# Autodesk Inventor assembly: Hilfsbaugruppe Vibrationsdämpfung
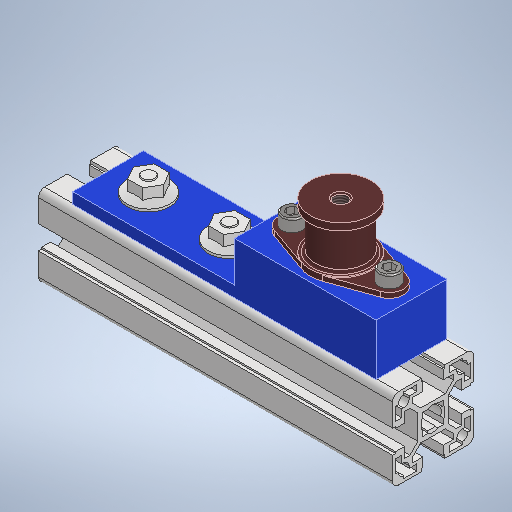
[picture p0: Inventor's stored thumbnail of the model, 512x512]
Saved by Autodesk Inventor 2025.2 (Build 292293000, 293)
## iProperties
Created: 2025-06-22
Part Number: Hilfsbaugruppe Vibrationsdämpfung
Document SubType Name: Assembly
Designer: Jakob
Author: Jakob
## Documents named in this file (6)
- D:\Useless_Box\CAD-Paspa\Useless Box\Zeichnung_JH\Hilfsbaugruppe Vibrationsdämpfung.iam
- D:\Useless_Box\CAD-Paspa\Useless Box\Eigene Bauteile\Vibrationsdaempfer\Rexroth_Profil_40x40_2175_8.ipt
- D:\Useless_Box\CAD-Paspa\Useless Box\Eigene Bauteile\Vibrationsdaempfer\Adapterplatte_Vibrationsdaempfer.ipt
- D:\Useless_Box\CAD-Paspa\Useless Box\Eigene Bauteile\Vibrationsdaempfer\AIS2024\NHF19-3026-M8.ipt
- D:\Useless_Box\CAD-Paspa\Useless Box\Standart Bauteile\ISO 4762 - M6 x 12ISO.ipt
- D:\Useless_Box\CAD-Paspa\Useless Box\Eigene Bauteile\Vibrationsdaempfer\Rexroth_Schraube_Mutter_modifiziert_fuer_daempfer.iam
## Components (7 placed, 5 different names)
1. Rexroth_Profil_40x40_2175_8:1 — Passend:1, Passend:2, Fluchtend:1, Fluchtend:4, Passend:10
2. Adapterplatte_Vibrationsdaempfer:1 — Passend:7, Fluchtend:4, Fluchtend:6, Passend:8, Passend:9, Passend:19, Passend:20, Fluchtend:7, Passend:21, Passend:22, Passend:23
3. NHF19-3026-M8:1 — Fluchtend:6, Passend:8, Passend:9, Passend:10, Passend:11, Passend:12, Passend:13, Passend:14
4. ISO 4762 - M6 x 12ISO:1 — Passend:12, Passend:14
5. ISO 4762 - M6 x 12ISO:2 — Passend:11, Passend:13
6. Rexroth_Schraube_Mutter_modifiziert_fuer_daempfer:1 [sub-assembly] — Fluchtend:7, Passend:21, Passend:23
7. Rexroth_Schraube_Mutter_modifiziert_fuer_daempfer:2 [sub-assembly] — Passend:19, Passend:20, Passend:22
## Relationships (19: Mate 15, Flush 4)
- Passend:1 [Mate]: Rexroth_Profil_40x40_2175_8:1
- Passend:2 [Mate]: Rexroth_Profil_40x40_2175_8:1
- Fluchtend:1 [Flush]: Rexroth_Profil_40x40_2175_8:1
- Passend:7 [Mate]: Adapterplatte_Vibrationsdaempfer:1
- Fluchtend:4 [Flush]: Rexroth_Profil_40x40_2175_8:1 ↔ Adapterplatte_Vibrationsdaempfer:1
- Fluchtend:6 [Flush]: Adapterplatte_Vibrationsdaempfer:1 ↔ NHF19-3026-M8:1
- Passend:8 [Mate]: Adapterplatte_Vibrationsdaempfer:1 ↔ NHF19-3026-M8:1
- Passend:9 [Mate]: Adapterplatte_Vibrationsdaempfer:1 ↔ NHF19-3026-M8:1
- Passend:10 [Mate] (45.642 mm): Rexroth_Profil_40x40_2175_8:1 ↔ NHF19-3026-M8:1
- Passend:11 [Mate]: NHF19-3026-M8:1 ↔ ISO 4762 - M6 x 12ISO:2
- Passend:12 [Mate]: NHF19-3026-M8:1 ↔ ISO 4762 - M6 x 12ISO:1
- Passend:13 [Mate]: NHF19-3026-M8:1 ↔ ISO 4762 - M6 x 12ISO:2
- Passend:14 [Mate]: NHF19-3026-M8:1 ↔ ISO 4762 - M6 x 12ISO:1
- Passend:19 [Mate]: Adapterplatte_Vibrationsdaempfer:1 ↔ Rexroth_Schraube_Mutter_modifiziert_fuer_daempfer:2
- Passend:20 [Mate]: Adapterplatte_Vibrationsdaempfer:1 ↔ Rexroth_Schraube_Mutter_modifiziert_fuer_daempfer:2
- Fluchtend:7 [Flush]: Adapterplatte_Vibrationsdaempfer:1 ↔ Rexroth_Schraube_Mutter_modifiziert_fuer_daempfer:1
- Passend:21 [Mate]: Adapterplatte_Vibrationsdaempfer:1 ↔ Rexroth_Schraube_Mutter_modifiziert_fuer_daempfer:1
- Passend:22 [Mate]: Adapterplatte_Vibrationsdaempfer:1 ↔ Rexroth_Schraube_Mutter_modifiziert_fuer_daempfer:2
- Passend:23 [Mate]: Adapterplatte_Vibrationsdaempfer:1 ↔ Rexroth_Schraube_Mutter_modifiziert_fuer_daempfer:1
